# Autodesk Inventor assembly: STARduino and Pi assembly
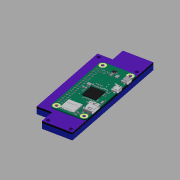
[picture p0: Inventor's stored thumbnail of the model, 180x180]
Saved by Autodesk Inventor 2017 (Build 210142000, 142)
## iProperties
Created: 2017-01-16
Part Number: STARduino and Pi assembly
Document SubType Name: Assembly
Designer: qupec
Author: qupec
## Documents named in this file (5)
- C:\Users\qupec\Desktop\UMD Near Space\RockSat\STARduino and Pi assembly.iam
- C:\Users\qupec\Desktop\UMD Near Space\RockSat\STARduino layout.ipt
- C:\Users\qupec\Desktop\UMD Near Space\RockSat\Pi Holder Mk2.ipt
- C:\Users\qupec\Desktop\UMD Near Space\RockSat\STARduino Mount.ipt
- C:\Users\qupec\Desktop\UMD Near Space\RockSat\Pi Cam\RapberryPiZero.ipt
## Components (4 placed, 4 different names)
1. STARduino layout:1 — Mate:7, Mate:8, Flush:2, Flush:3, Mate:11, Mate:12
2. Pi Holder Mk2:1 — Mate:9, Flush:4, Mate:10, Mate:11, Mate:12
3. STARduino Mount:1 — Mate:7, Mate:9, Flush:4, Mate:10
4. RapberryPiZero:1 — Mate:8, Flush:2, Flush:3
## Relationships (9: Mate 6, Flush 3)
- Mate:7: STARduino layout:1 ↔ STARduino Mount:1
- Mate:8: STARduino layout:1 ↔ RapberryPiZero:1
- Flush:2 (16.51 mm): STARduino layout:1 ↔ RapberryPiZero:1
- Flush:3: STARduino layout:1 ↔ RapberryPiZero:1
- Mate:9: Pi Holder Mk2:1 ↔ STARduino Mount:1
- Flush:4: Pi Holder Mk2:1 ↔ STARduino Mount:1
- Mate:10: Pi Holder Mk2:1 ↔ STARduino Mount:1
- Mate:11: STARduino layout:1 ↔ Pi Holder Mk2:1
- Mate:12: STARduino layout:1 ↔ Pi Holder Mk2:1
